# Autodesk Inventor assembly: DRIVETRAIN,ELEVATOR
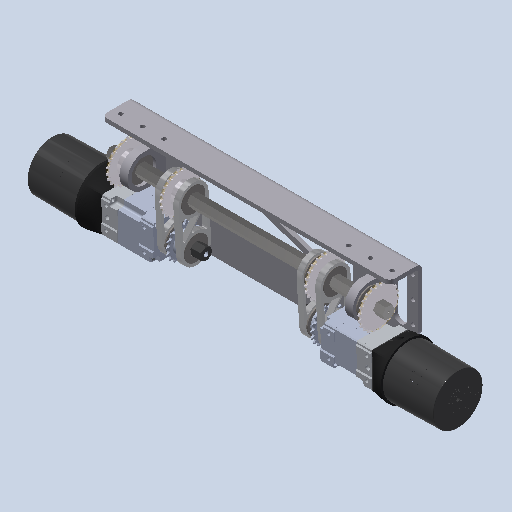
[picture p0: Inventor's stored thumbnail of the model, 512x512]
Saved by Autodesk Inventor 2025.2 (Build 292293000, 293)
## iProperties
Category: _
Manager: _
Created: 2025-03-14
Part Number: DRIVETRAIN,ELEVATOR
Checked By: 00
Engr Approved By: _
User Status: Work In Process
Description: ASSY,STANDARD (mm)
Document SubType Name: Assembly
Mfg Approved By: -
Designer: John Thibert
CN_MASS: 0.0
CN_SERVICEABLE: _
FIRST_DESCRIPTION: _
SECOND_DESCRIPTION: _
THIRD_DESCRIPTION: _
CL_runCount: 0
ModelCat: Uncategorized
ILogicPurgeVersion: 3.4.1.0
ILogicPurgeAssembly: InventorDocumentWrapper
Subject: _
Author: John Thibert
Keywords: -
Revision Number: A
## Documents named in this file (12)
- C:\Users\Baz Robotics\Downloads\2025-Poseidon-Mechanical\DRIVETRAIN,ELEVATOR.iam
- C:\Users\Baz Robotics\Downloads\2025-Poseidon-Mechanical\22.ipt
- C:\Users\Baz Robotics\Downloads\2025-Poseidon-Mechanical\PLATE,MOUNT,DRIVE,ELEVATOR.ipt
- C:\Users\Baz Robotics\Downloads\2025-Poseidon-Mechanical\PLATE,BEARING,DRIVE,ELEVATOR.ipt
- C:\Users\Baz Robotics\Downloads\2025-Poseidon-Mechanical\PURCHASED,HEX_BEARING.ipt
- C:\Users\Baz Robotics\Downloads\2025-Poseidon-Mechanical\SHAFT,HEX,0.500in,DRIVE,ELEVATOR.ipt
- C:\Users\Baz Robotics\Downloads\2025-Poseidon-Mechanical\VersaPlanetary v2 Dual Stage 10_1 with RS 550 (1).iam
- C:\Users\Baz Robotics\Downloads\2025-Poseidon-Mechanical\BRACE,SHAFT,ELEVATOR.ipt
- C:\Users\Baz Robotics\Downloads\2025-Poseidon-Mechanical\WCP-0754.ipt
- C:\Users\Baz Robotics\Downloads\2025-Poseidon-Mechanical\SPACER,HEX,0.125IN.ipt
- C:\Users\Baz Robotics\Downloads\2025-Poseidon-Mechanical\CONTROLS,MOTOR,NEO,V1.ipt
- C:\Users\Baz Robotics\Downloads\2025-Poseidon-Mechanical\1_CAD Library\PURCHASED,GEARBOX,VERSA_PLANETARY,ADAPTER_CIM.ipt
## Components (33 placed, 13 different names)
1. CONTROLS,MOTOR,NEO,V1:1
2. PURCHASED,GEARBOX,VERSA_PLANETARY,ADAPTER_CIM:1
3. BRACE,SHAFT,ELEVATOR:1
4. WCP-0754:1
5. PURCHASED,HEX_BEARING:3
6. PURCHASED,HEX_BEARING:5
7. BRACE,SHAFT,ELEVATOR:2
8. VersaPlanetary v2 Dual Stage 10_1 with RS 550 (1):1 [sub-assembly]
9. SHAFT,HEX,0.500in,DRIVE,ELEVATOR.ipt:1
10. 22:3
11. 22.ipt:2
12. PURCHASED,HEX_BEARING.ipt:1
13. PLATE,BEARING,DRIVE,ELEVATOR.ipt:2
14. PLATE,MOUNT,DRIVE,ELEVATOR.ipt:1
15. PURCHASED,HEX_BEARING:4
16. SPACER,HEX,0.125IN:1
17. PURCHASED,HEX_BEARING:6
18. BRACE,SHAFT,ELEVATOR:3
19. PURCHASED,HEX_BEARING:8
20. 22:4
21. SPACER,HEX,0.125IN:3
22. PURCHASED,HEX_BEARING:10
23. BRACE,SHAFT,ELEVATOR:4
24. WCP-0754:2
25. PURCHASED,HEX_BEARING:7
26. SPACER,HEX,0.125IN:2
27. PURCHASED,HEX_BEARING:9
28. VersaPlanetary v2 Dual Stage 10_1 with RS 550 (1):2 [sub-assembly]
29. PLATE,BEARING,DRIVE,ELEVATOR.ipt:1
30. PURCHASED,HEX_BEARING.ipt:2
31. 22.ipt:1
32. PURCHASED,GEARBOX,VERSA_PLANETARY,ADAPTER_CIM:2
33. CONTROLS,MOTOR,NEO,V1:2
## Relationships (64: Mate 45, Insert 12, Angle 4, Flush 3)
- [Mate]: PLATE,MOUNT,DRIVE,ELEVATOR.ipt:1 ↔ PLATE,BEARING,DRIVE,ELEVATOR.ipt:1
- [Mate]: PLATE,BEARING,DRIVE,ELEVATOR.ipt:1 ↔ 22.ipt:1
- [Mate]: PLATE,MOUNT,DRIVE,ELEVATOR.ipt:1 ↔ PLATE,BEARING,DRIVE,ELEVATOR.ipt:1
- [Mate]: PLATE,MOUNT,DRIVE,ELEVATOR.ipt:1 ↔ PLATE,BEARING,DRIVE,ELEVATOR.ipt:1
- [Mate]: PLATE,BEARING,DRIVE,ELEVATOR.ipt:2 ↔ PLATE,MOUNT,DRIVE,ELEVATOR.ipt:1
- [Mate]: PLATE,BEARING,DRIVE,ELEVATOR.ipt:2 ↔ PLATE,MOUNT,DRIVE,ELEVATOR.ipt:1
- [Mate]: PLATE,BEARING,DRIVE,ELEVATOR.ipt:2 ↔ PLATE,MOUNT,DRIVE,ELEVATOR.ipt:1
- [Insert]: PURCHASED,HEX_BEARING.ipt:1 ↔ PLATE,BEARING,DRIVE,ELEVATOR.ipt:2
- [Insert]: PLATE,BEARING,DRIVE,ELEVATOR.ipt:1 ↔ PURCHASED,HEX_BEARING.ipt:2
- [Mate]: 22.ipt:2 ↔ PLATE,BEARING,DRIVE,ELEVATOR.ipt:2
- [Mate]: SHAFT,HEX,0.500in,DRIVE,ELEVATOR.ipt:1 ↔ PLATE,BEARING,DRIVE,ELEVATOR.ipt:2
- [Angle] (0 deg): SHAFT,HEX,0.500in,DRIVE,ELEVATOR.ipt:1 ↔ 22.ipt:2
- [Angle] (0 deg): SHAFT,HEX,0.500in,DRIVE,ELEVATOR.ipt:1 ↔ PURCHASED,HEX_BEARING.ipt:1
- [Angle] (0 deg): SHAFT,HEX,0.500in,DRIVE,ELEVATOR.ipt:1 ↔ 22.ipt:1
- [Angle] (0 deg): SHAFT,HEX,0.500in,DRIVE,ELEVATOR.ipt:1 ↔ PURCHASED,HEX_BEARING.ipt:2
- [Flush] (-15.875 mm): SHAFT,HEX,0.500in,DRIVE,ELEVATOR.ipt:1 ↔ 22.ipt:2
- [Mate]: PLATE,MOUNT,DRIVE,ELEVATOR.ipt:1 ↔ VersaPlanetary v2 Dual Stage 10_1 with RS 550 (1):2
- [Mate]: BRACE,SHAFT,ELEVATOR:1 ↔ VersaPlanetary v2 Dual Stage 10_1 with RS 550 (1):1
- [Insert]: BRACE,SHAFT,ELEVATOR:1 ↔ PURCHASED,HEX_BEARING:4
- [Insert]: BRACE,SHAFT,ELEVATOR:1 ↔ PURCHASED,HEX_BEARING:3
- [Mate]: PURCHASED,HEX_BEARING:3 ↔ VersaPlanetary v2 Dual Stage 10_1 with RS 550 (1):1
- [Insert]: BRACE,SHAFT,ELEVATOR:2 ↔ PURCHASED,HEX_BEARING:6
- [Insert]: PURCHASED,HEX_BEARING:5 ↔ BRACE,SHAFT,ELEVATOR:2
- [Mate]: BRACE,SHAFT,ELEVATOR:2 ↔ VersaPlanetary v2 Dual Stage 10_1 with RS 550 (1):1
- [Mate]: BRACE,SHAFT,ELEVATOR:1 ↔ BRACE,SHAFT,ELEVATOR:2
- [Mate]: WCP-0754:1 ↔ VersaPlanetary v2 Dual Stage 10_1 with RS 550 (1):1
- [Flush]: WCP-0754:1 ↔ 22:3
- [Mate]: 22:3 ↔ PURCHASED,HEX_BEARING:6
- [Mate]: PURCHASED,HEX_BEARING:4 ↔ SPACER,HEX,0.125IN:1
- [Mate]: BRACE,SHAFT,ELEVATOR:1 ↔ SPACER,HEX,0.125IN:1
- [Mate]: 22:3 ↔ SPACER,HEX,0.125IN:1
- [Insert]: BRACE,SHAFT,ELEVATOR:3 ↔ PURCHASED,HEX_BEARING:8
- [Insert]: BRACE,SHAFT,ELEVATOR:3 ↔ PURCHASED,HEX_BEARING:7
- [Insert]: PURCHASED,HEX_BEARING:10 ↔ BRACE,SHAFT,ELEVATOR:4
- [Insert]: BRACE,SHAFT,ELEVATOR:4 ↔ PURCHASED,HEX_BEARING:9
- [Mate]: BRACE,SHAFT,ELEVATOR:3 ↔ BRACE,SHAFT,ELEVATOR:4
- [Flush]: 22:4 ↔ WCP-0754:2
- [Mate]: SPACER,HEX,0.125IN:3 ↔ PURCHASED,HEX_BEARING:10
- [Mate]: BRACE,SHAFT,ELEVATOR:3 ↔ SPACER,HEX,0.125IN:3
- [Mate]: 22:4 ↔ SPACER,HEX,0.125IN:3
- [Mate]: BRACE,SHAFT,ELEVATOR:4 ↔ VersaPlanetary v2 Dual Stage 10_1 with RS 550 (1):2
- [Mate]: BRACE,SHAFT,ELEVATOR:3 ↔ VersaPlanetary v2 Dual Stage 10_1 with RS 550 (1):2
- [Mate]: BRACE,SHAFT,ELEVATOR:3 ↔ SPACER,HEX,0.125IN:2
- [Mate]: SPACER,HEX,0.125IN:2 ↔ PURCHASED,HEX_BEARING:9
- [Mate]: WCP-0754:2 ↔ SPACER,HEX,0.125IN:2
- [Mate]: 22:4 ↔ BRACE,SHAFT,ELEVATOR:4
- [Mate]: BRACE,SHAFT,ELEVATOR:4 ↔ WCP-0754:2
- [Mate]: PURCHASED,HEX_BEARING:9 ↔ VersaPlanetary v2 Dual Stage 10_1 with RS 550 (1):2
- [Mate]: WCP-0754:2 ↔ PURCHASED,HEX_BEARING:7
- [Mate]: BRACE,SHAFT,ELEVATOR:2 ↔ BRACE,SHAFT,ELEVATOR:3
- [Insert]: CONTROLS,MOTOR,NEO,V1:1 ↔ PURCHASED,GEARBOX,VERSA_PLANETARY,ADAPTER_CIM:1
- [Insert]: PURCHASED,GEARBOX,VERSA_PLANETARY,ADAPTER_CIM:2 ↔ CONTROLS,MOTOR,NEO,V1:2
- [Mate]: VersaPlanetary v2 Dual Stage 10_1 with RS 550 (1):1 ↔ PLATE,MOUNT,DRIVE,ELEVATOR.ipt:1
- [Mate]: VersaPlanetary v2 Dual Stage 10_1 with RS 550 (1):1 ↔ VersaPlanetary v2 Dual Stage 10_1 with RS 550 (1):2
- [Mate]: PURCHASED,GEARBOX,VERSA_PLANETARY,ADAPTER_CIM:1 ↔ VersaPlanetary v2 Dual Stage 10_1 with RS 550 (1):1
- [Mate]: VersaPlanetary v2 Dual Stage 10_1 with RS 550 (1):2 ↔ PURCHASED,GEARBOX,VERSA_PLANETARY,ADAPTER_CIM:2
- [Mate]: VersaPlanetary v2 Dual Stage 10_1 with RS 550 (1):2 ↔ CONTROLS,MOTOR,NEO,V1:2
- [Mate]: CONTROLS,MOTOR,NEO,V1:1 ↔ VersaPlanetary v2 Dual Stage 10_1 with RS 550 (1):1
- [Mate]: VersaPlanetary v2 Dual Stage 10_1 with RS 550 (1):1 ↔ PLATE,MOUNT,DRIVE,ELEVATOR.ipt:1
- [Mate]: PLATE,MOUNT,DRIVE,ELEVATOR.ipt:1 ↔ VersaPlanetary v2 Dual Stage 10_1 with RS 550 (1):2
- [Mate]: VersaPlanetary v2 Dual Stage 10_1 with RS 550 (1):2 ↔ PURCHASED,GEARBOX,VERSA_PLANETARY,ADAPTER_CIM:2
- [Mate]: PURCHASED,GEARBOX,VERSA_PLANETARY,ADAPTER_CIM:2 ↔ CONTROLS,MOTOR,NEO,V1:2
- [Mate]: CONTROLS,MOTOR,NEO,V1:1 ↔ PURCHASED,GEARBOX,VERSA_PLANETARY,ADAPTER_CIM:1
- [Mate]: PURCHASED,GEARBOX,VERSA_PLANETARY,ADAPTER_CIM:1 ↔ VersaPlanetary v2 Dual Stage 10_1 with RS 550 (1):1
## Named parameters: d1144_d1133 = 0 mm, d1145_d1134 = 0 mm, d1176_d1175 = 0 mm, d1116_d1113 = 0 mm, d1117_d1114 = 0 mm, d1135_d1113 = 0 mm, d1136_d1114 = 0 mm, d1137_d1116_d1113 = 0 mm, d1138_d1117_d1114 = 0 mm, d1139_d1123 = 0 mm, d1140_d1127 = 0 mm, d1143_d1132 = 0 mm
